# Autodesk Inventor assembly: elevation_assembly_blacha_gieta
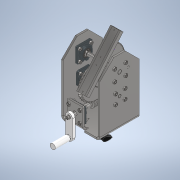
[picture p0: Inventor's stored thumbnail of the model, 180x180]
Saved by Autodesk Inventor 2020 (Build 240168000, 168)
## iProperties
Created: 2020-08-26
Part Number: elevation_assembly_blacha_gieta
Document SubType Name: Assembly
Designer: Hesekiel
Author: Hesekiel
## Documents named in this file (43)
- C:\Users\Hesekiel\Desktop\Equatorial-Mount-MUM\Mechanika\Mechanizm elewacji Filip\CAD\elevation_assembly_blacha_gieta.iam
- C:\Users\Hesekiel\Desktop\Equatorial-Mount-MUM\Mechanika\Mechanizm elewacji Filip\CAD\baza_blacha_gięta.ipt
- C:\Users\Hesekiel\Desktop\Equatorial-Mount-MUM\Mechanika\Mechanizm elewacji Filip\CAD\F4BSS 20M-YTPSS\F4BSS 20M-YTPSS.iam
- C:\Users\Hesekiel\Desktop\Equatorial-Mount-MUM\Mechanika\Mechanizm elewacji Filip\CAD\FY 15 FM\FY 15 FM.iam
- C:\Users\Hesekiel\Desktop\Equatorial-Mount-MUM\Mechanika\Mechanizm elewacji Filip\CAD\elevation_assembly_blacha_gieta\Design Accelerator\Bolted Connection4.iam
- C:\Users\Hesekiel\Desktop\Equatorial-Mount-MUM\Mechanika\Mechanizm elewacji Filip\CAD\elevation_assembly_blacha_gieta\Design Accelerator\Bolted Connection5.iam
- C:\Users\Hesekiel\Desktop\Equatorial-Mount-MUM\Mechanika\Mechanizm elewacji Filip\CAD\elevation_assembly_blacha_gieta\Design Accelerator\Bolted Connection6.iam
- C:\Users\Hesekiel\Desktop\Equatorial-Mount-MUM\Mechanika\Mechanizm elewacji Filip\CAD\elevation_assembly_blacha_gieta\Design Accelerator\Bolted Connection7.iam
- C:\Users\Hesekiel\Desktop\Equatorial-Mount-MUM\Mechanika\Mechanizm elewacji Filip\CAD\elevation_assembly_blacha_gieta\Design Accelerator\Bolted Connection8.iam
- C:\Users\Hesekiel\Desktop\Equatorial-Mount-MUM\Mechanika\Mechanizm elewacji Filip\CAD\elevation_assembly_blacha_gieta\Design Accelerator\Bolted Connection9.iam
- C:\Users\Hesekiel\Desktop\Equatorial-Mount-MUM\Mechanika\Mechanizm elewacji Filip\CAD\elevation_assembly_blacha_gieta\Design Accelerator\Bolted Connection10.iam
- C:\Users\Hesekiel\Desktop\Equatorial-Mount-MUM\Mechanika\Mechanizm elewacji Filip\CAD\elevation_assembly_blacha_gieta\Design Accelerator\Bolted Connection11.iam
- C:\Users\Hesekiel\Desktop\Equatorial-Mount-MUM\Mechanika\Mechanizm elewacji Filip\CAD\elevation_assembly_blacha_gieta\Design Accelerator\Bolted Connection12.iam
- C:\Users\Hesekiel\Desktop\Equatorial-Mount-MUM\Mechanika\Mechanizm elewacji Filip\CAD\elevation_assembly_blacha_gieta\Design Accelerator\Bolted Connection13.iam
- C:\Users\Hesekiel\Desktop\Equatorial-Mount-MUM\Mechanika\Mechanizm elewacji Filip\CAD\elevation_assembly_blacha_gieta\Design Accelerator\Bolted Connection14.iam
- C:\Users\Hesekiel\Desktop\Equatorial-Mount-MUM\Mechanika\Mechanizm elewacji Filip\CAD\elevation_assembly_blacha_gieta\Design Accelerator\Bolted Connection15.iam
- C:\Users\Hesekiel\Desktop\Equatorial-Mount-MUM\Mechanika\Mechanizm elewacji Filip\CAD\elevation_assembly_blacha_gieta\Design Accelerator\Bolted Connection16.iam
- C:\Users\Hesekiel\Desktop\Equatorial-Mount-MUM\Mechanika\Mechanizm elewacji Filip\CAD\elevation_assembly_blacha_gieta\Design Accelerator\Bolted Connection17.iam
- C:\Users\Hesekiel\Desktop\Equatorial-Mount-MUM\Mechanika\Mechanizm elewacji Filip\CAD\elevation_assembly_blacha_gieta\Design Accelerator\Bolted Connection18.iam
- C:\Users\Hesekiel\Desktop\Equatorial-Mount-MUM\Mechanika\Mechanizm elewacji Filip\CAD\elevation_assembly_blacha_gieta\Design Accelerator\Bolted Connection19.iam
- C:\Users\Hesekiel\Desktop\Equatorial-Mount-MUM\Mechanika\Mechanizm elewacji Filip\CAD\elevation_assembly_blacha_gieta\Design Accelerator\Bolted Connection20.iam
- C:\Users\Hesekiel\Desktop\Equatorial-Mount-MUM\Mechanika\Mechanizm elewacji Filip\CAD\elevation_assembly_blacha_gieta\Design Accelerator\Bolted Connection21.iam
- C:\Users\Hesekiel\Desktop\Equatorial-Mount-MUM\Mechanika\Mechanizm elewacji Filip\CAD\elevation_assembly_blacha_gieta\Design Accelerator\Bolted Connection22.iam
- C:\Users\Hesekiel\Desktop\Equatorial-Mount-MUM\Mechanika\Mechanizm elewacji Filip\CAD\elevation_assembly_blacha_gieta\Design Accelerator\Bolted Connection23.iam
- C:\Users\Hesekiel\Desktop\Equatorial-Mount-MUM\Mechanika\Mechanizm elewacji Filip\CAD\elevation_assembly_blacha_gieta\Design Accelerator\Bolted Connection24.iam
- C:\Users\Hesekiel\Desktop\Equatorial-Mount-MUM\Mechanika\Mechanizm elewacji Filip\CAD\elevation_assembly_blacha_gieta\Design Accelerator\Bolted Connection25.iam
- C:\Users\Hesekiel\Desktop\Equatorial-Mount-MUM\Mechanika\Mechanizm elewacji Filip\CAD\elevation_assembly_blacha_gieta\Design Accelerator\Bolted Connection26.iam
- C:\Users\Hesekiel\Desktop\Equatorial-Mount-MUM\Mechanika\Mechanizm elewacji Filip\CAD\elevation_assembly_blacha_gieta\Design Accelerator\Bolted Connection27.iam
- C:\Users\Hesekiel\Desktop\Equatorial-Mount-MUM\Mechanika\Mechanizm elewacji Filip\CAD\wał_półkola.ipt
- C:\Users\Hesekiel\Desktop\Equatorial-Mount-MUM\Mechanika\Mechanizm elewacji Filip\CAD\worm_gear.iam
- C:\Users\Hesekiel\Desktop\Equatorial-Mount-MUM\Mechanika\Mechanizm elewacji Filip\CAD\rack_and_pinion.iam
- C:\Users\Hesekiel\Desktop\Equatorial-Mount-MUM\Mechanika\Mechanizm elewacji Filip\CAD\wał_uzębienia.ipt
- C:\Users\Hesekiel\Desktop\Equatorial-Mount-MUM\Mechanika\Mechanizm elewacji Filip\CAD\ramię_korby.ipt
- C:\Users\Hesekiel\Desktop\Equatorial-Mount-MUM\Mechanika\Mechanizm elewacji Filip\CAD\rączka_korby.ipt
- C:\Users\Hesekiel\Desktop\Equatorial-Mount-MUM\Mechanika\Mechanizm elewacji Filip\CAD\elevation_assembly_blacha_gieta\Design Accelerator\Bolted Connection28.iam
- C:\Users\Hesekiel\Desktop\Equatorial-Mount-MUM\Mechanika\Mechanizm elewacji Filip\CAD\elevation_assembly_blacha_gieta\Design Accelerator\Bolted Connection29.iam
- C:\Users\Hesekiel\Desktop\Equatorial-Mount-MUM\Mechanika\Uchwyty, elementy i inne\szyna.ipt
- C:\Users\Hesekiel\Desktop\Equatorial-Mount-MUM\Mechanika\Mechanizm elewacji Filip\CAD\uchwyt_szyny.ipt
- C:\Users\Hesekiel\Desktop\Equatorial-Mount-MUM\Mechanika\Mechanizm elewacji Filip\CAD\elevation_assembly_blacha_gieta\Design Accelerator\Bolted Connection31.iam
- C:\Users\Hesekiel\Desktop\Equatorial-Mount-MUM\Mechanika\Mechanizm elewacji Filip\CAD\elevation_assembly_blacha_gieta\Design Accelerator\Bolted Connection32.iam
- C:\Users\Hesekiel\Desktop\Equatorial-Mount-MUM\Mechanika\Mechanizm elewacji Filip\CAD\elevation_assembly_blacha_gieta\Design Accelerator\Bolted Connection33.iam
- C:\Users\Hesekiel\Desktop\Equatorial-Mount-MUM\Mechanika\Mechanizm elewacji Filip\CAD\manfrotto-494rc2-tripod-head.snapshot.1\Manfrotto 494RC2 - Tripod Head\Manfrotto - 494RC2 Head Assy.iam
- C:\Users\Hesekiel\Desktop\Equatorial-Mount-MUM\Mechanika\Mechanizm elewacji Filip\CAD\M6x6_DIN914.ipt
## Components (48 placed, 14 different names)
1. baza_blacha_gięta:1 — Flush:1, Mate:1, Mate:2, Mate:3, Mate:4, Mate:5, Mate:6, Mate:7, Mate:21, Mate:22, Mate:23, Mate:24, Mate:25, Mate:26, Mate:27, Mate:28, Mate:29, Mate:30, Mate:31, Mate:32, Rotational:2, Angle:1, Rotational:3, Angle:2, Rotational:4, Mate:101, Mate:102
2. F4BSS 20M-YTPSS:1 [sub-assembly] — Mate:2, Mate:3, Mate:4, Mate:57, Mate:58, Mate:59, Mate:60, Mate:61, Mate:62, Mate:63, Mate:64
3. F4BSS 20M-YTPSS:2 [sub-assembly] — Mate:5, Mate:6, Mate:7, Mate:49, Mate:50, Mate:51, Mate:52, Mate:53, Mate:54, Mate:55, Mate:56
4. FY 15 FM:1 [sub-assembly] — Mate:21, Mate:22, Mate:23, Mate:41, Mate:42, Mate:43, Mate:44, Mate:45, Mate:46, Mate:47, Mate:48
5. FY 15 FM:2 [sub-assembly] — Mate:24, Mate:25, Mate:26, Mate:73, Mate:74, Mate:75, Mate:76, Mate:77, Mate:78, Mate:79, Mate:80
6. F4BSS 20M-YTPSS:3 [sub-assembly] — Mate:30, Mate:31, Mate:32, Mate:65, Mate:66, Mate:67, Mate:68, Mate:69, Mate:70, Mate:71, Mate:72
7. F4BSS 20M-YTPSS:4 [sub-assembly] — Mate:27, Mate:28, Mate:29, Mate:33, Mate:34, Mate:35, Mate:36, Mate:37, Mate:38, Mate:39, Mate:40
8. Bolted Connection:1 [sub-assembly] — Mate:33, Mate:34
9. Bolted Connection:2 [sub-assembly] — Mate:35, Mate:36
10. Bolted Connection:3 [sub-assembly] — Mate:37, Mate:38
11. Bolted Connection:4 [sub-assembly] — Mate:39, Mate:40
12. Bolted Connection:5 [sub-assembly] — Mate:41, Mate:42
13. Bolted Connection:6 [sub-assembly] — Mate:43, Mate:44
14. Bolted Connection:7 [sub-assembly] — Mate:45, Mate:46
15. Bolted Connection:8 [sub-assembly] — Mate:47, Mate:48
16. Bolted Connection:9 [sub-assembly] — Mate:49, Mate:50
17. Bolted Connection:10 [sub-assembly] — Mate:51, Mate:52
18. Bolted Connection:11 [sub-assembly] — Mate:53, Mate:54
19. Bolted Connection:12 [sub-assembly] — Mate:55, Mate:56
20. Bolted Connection:13 [sub-assembly] — Mate:57, Mate:58
21. Bolted Connection:14 [sub-assembly] — Mate:59, Mate:60
22. Bolted Connection:15 [sub-assembly] — Mate:61, Mate:62
23. Bolted Connection:16 [sub-assembly] — Mate:63, Mate:64
24. Bolted Connection:17 [sub-assembly] — Mate:65, Mate:66
25. Bolted Connection:18 [sub-assembly] — Mate:67, Mate:68
26. Bolted Connection:19 [sub-assembly] — Mate:69, Mate:70
27. Bolted Connection:20 [sub-assembly] — Mate:71, Mate:72
28. Bolted Connection:21 [sub-assembly] — Mate:73, Mate:74
29. Bolted Connection:22 [sub-assembly] — Mate:75, Mate:76
30. Bolted Connection:23 [sub-assembly] — Mate:77, Mate:78
31. Bolted Connection:24 [sub-assembly] — Mate:79, Mate:80
32. wał_półkola:1 — Rotational:2, Angle:1, Mate:81, Mate:107
33. rack_and_pinion:1 [sub-assembly] — Mate:81, Mate:82, Mate:84, Mate:92, Mate:93, Mate:94, Mate:104, Mate:108
34. worm_gear:1 [sub-assembly] — Mate:83, Mate:84, Rotational:4, Rigid:6, Mate:106
35. wał_uzębienia:1 — Rotational:3, Angle:2, Mate:82, Mate:83, Mate:103, Mate:105
36. ramię_korby:1 — Rigid:6, Rigid:7, Mate:85, Mate:86, Mate:87, Mate:88
37. rączka_korby:1 — Rigid:7
38. Bolted Connection:25 [sub-assembly] — Mate:85, Mate:86
39. Bolted Connection:26 [sub-assembly] — Mate:87, Mate:88
40. uchwyt_szyny:1 — Flush:2, Mate:89, Mate:90, Mate:91, Mate:92, Mate:93, Mate:94, Mate:95, Mate:96, Mate:97, Mate:98, Mate:99, Mate:100
41. Bolted Connection:27 [sub-assembly] — Mate:95, Mate:96
42. Bolted Connection:28 [sub-assembly] — Mate:97, Mate:98
43. Bolted Connection:29 [sub-assembly] — Mate:99, Mate:100
44. szyna:1 — Flush:2, Mate:89, Mate:90, Mate:91
45. Manfrotto - 494RC2 Head Assy:1 [sub-assembly] — Mate:101, Mate:102
46. M6x6_DIN914:1 — Mate:103, Mate:104
47. M6x6_DIN914:2 — Mate:105, Mate:106
48. M6x6_DIN914:3 — Mate:107, Mate:108
## Relationships (104: Mate 95, RevoluteJoint 3, Flush 2, Angle 2, WeldJoint 2)
- Flush:1: baza_blacha_gięta:1
- Mate:1: baza_blacha_gięta:1
- Mate:2: baza_blacha_gięta:1 ↔ F4BSS 20M-YTPSS:1
- Mate:3: baza_blacha_gięta:1 ↔ F4BSS 20M-YTPSS:1
- Mate:4: baza_blacha_gięta:1 ↔ F4BSS 20M-YTPSS:1
- Mate:5: baza_blacha_gięta:1 ↔ F4BSS 20M-YTPSS:2
- Mate:6: baza_blacha_gięta:1 ↔ F4BSS 20M-YTPSS:2
- Mate:7: baza_blacha_gięta:1 ↔ F4BSS 20M-YTPSS:2
- Mate:21: baza_blacha_gięta:1 ↔ FY 15 FM:1
- Mate:22: baza_blacha_gięta:1 ↔ FY 15 FM:1
- Mate:23: baza_blacha_gięta:1 ↔ FY 15 FM:1
- Mate:24: baza_blacha_gięta:1 ↔ FY 15 FM:2
- Mate:25: baza_blacha_gięta:1 ↔ FY 15 FM:2
- Mate:26: baza_blacha_gięta:1 ↔ FY 15 FM:2
- Mate:27: baza_blacha_gięta:1 ↔ F4BSS 20M-YTPSS:4
- Mate:28: baza_blacha_gięta:1 ↔ F4BSS 20M-YTPSS:4
- Mate:29: baza_blacha_gięta:1 ↔ F4BSS 20M-YTPSS:4
- Mate:30: baza_blacha_gięta:1 ↔ F4BSS 20M-YTPSS:3
- Mate:31: baza_blacha_gięta:1 ↔ F4BSS 20M-YTPSS:3
- Mate:32: baza_blacha_gięta:1 ↔ F4BSS 20M-YTPSS:3
- Mate:33: F4BSS 20M-YTPSS:4 ↔ Bolted Connection:1
- Mate:34: F4BSS 20M-YTPSS:4 ↔ Bolted Connection:1
- Mate:35: F4BSS 20M-YTPSS:4 ↔ Bolted Connection:2
- Mate:36: F4BSS 20M-YTPSS:4 ↔ Bolted Connection:2
- Mate:37: F4BSS 20M-YTPSS:4 ↔ Bolted Connection:3
- Mate:38: F4BSS 20M-YTPSS:4 ↔ Bolted Connection:3
- Mate:39: F4BSS 20M-YTPSS:4 ↔ Bolted Connection:4
- Mate:40: F4BSS 20M-YTPSS:4 ↔ Bolted Connection:4
- Mate:41: FY 15 FM:1 ↔ Bolted Connection:5
- Mate:42: FY 15 FM:1 ↔ Bolted Connection:5
- Mate:43: FY 15 FM:1 ↔ Bolted Connection:6
- Mate:44: FY 15 FM:1 ↔ Bolted Connection:6
- Mate:45: FY 15 FM:1 ↔ Bolted Connection:7
- Mate:46: FY 15 FM:1 ↔ Bolted Connection:7
- Mate:47: FY 15 FM:1 ↔ Bolted Connection:8
- Mate:48: FY 15 FM:1 ↔ Bolted Connection:8
- Mate:49: F4BSS 20M-YTPSS:2 ↔ Bolted Connection:9
- Mate:50: F4BSS 20M-YTPSS:2 ↔ Bolted Connection:9
- Mate:51: F4BSS 20M-YTPSS:2 ↔ Bolted Connection:10
- Mate:52: F4BSS 20M-YTPSS:2 ↔ Bolted Connection:10
- Mate:53: F4BSS 20M-YTPSS:2 ↔ Bolted Connection:11
- Mate:54: F4BSS 20M-YTPSS:2 ↔ Bolted Connection:11
- Mate:55: F4BSS 20M-YTPSS:2 ↔ Bolted Connection:12
- Mate:56: F4BSS 20M-YTPSS:2 ↔ Bolted Connection:12
- Mate:57: F4BSS 20M-YTPSS:1 ↔ Bolted Connection:13
- Mate:58: F4BSS 20M-YTPSS:1 ↔ Bolted Connection:13
- Mate:59: F4BSS 20M-YTPSS:1 ↔ Bolted Connection:14
- Mate:60: F4BSS 20M-YTPSS:1 ↔ Bolted Connection:14
- Mate:61: F4BSS 20M-YTPSS:1 ↔ Bolted Connection:15
- Mate:62: F4BSS 20M-YTPSS:1 ↔ Bolted Connection:15
- Mate:63: F4BSS 20M-YTPSS:1 ↔ Bolted Connection:16
- Mate:64: F4BSS 20M-YTPSS:1 ↔ Bolted Connection:16
- Mate:65: F4BSS 20M-YTPSS:3 ↔ Bolted Connection:17
- Mate:66: F4BSS 20M-YTPSS:3 ↔ Bolted Connection:17
- Mate:67: F4BSS 20M-YTPSS:3 ↔ Bolted Connection:18
- Mate:68: F4BSS 20M-YTPSS:3 ↔ Bolted Connection:18
- Mate:69: F4BSS 20M-YTPSS:3 ↔ Bolted Connection:19
- Mate:70: F4BSS 20M-YTPSS:3 ↔ Bolted Connection:19
- Mate:71: F4BSS 20M-YTPSS:3 ↔ Bolted Connection:20
- Mate:72: F4BSS 20M-YTPSS:3 ↔ Bolted Connection:20
- Mate:73: FY 15 FM:2 ↔ Bolted Connection:21
- Mate:74: FY 15 FM:2 ↔ Bolted Connection:21
- Mate:75: FY 15 FM:2 ↔ Bolted Connection:22
- Mate:76: FY 15 FM:2 ↔ Bolted Connection:22
- Mate:77: FY 15 FM:2 ↔ Bolted Connection:23
- Mate:78: FY 15 FM:2 ↔ Bolted Connection:23
- Mate:79: FY 15 FM:2 ↔ Bolted Connection:24
- Mate:80: FY 15 FM:2 ↔ Bolted Connection:24
- Rotational:2 [RevoluteJoint]: baza_blacha_gięta:1 ↔ wał_półkola:1
- Angle:1 (0 deg): baza_blacha_gięta:1 ↔ wał_półkola:1
- Rotational:3 [RevoluteJoint]: baza_blacha_gięta:1 ↔ wał_uzębienia:1
- Angle:2 (0 deg): baza_blacha_gięta:1 ↔ wał_uzębienia:1
- Mate:81: wał_półkola:1 ↔ rack_and_pinion:1
- Mate:82: rack_and_pinion:1 ↔ wał_uzębienia:1
- Mate:83: worm_gear:1 ↔ wał_uzębienia:1
- Mate:84 (10 mm): rack_and_pinion:1 ↔ worm_gear:1
- Rotational:4 [RevoluteJoint]: baza_blacha_gięta:1 ↔ worm_gear:1
- Rigid:6 [WeldJoint]: worm_gear:1 ↔ ramię_korby:1
- Rigid:7 [WeldJoint]: ramię_korby:1 ↔ rączka_korby:1
- Mate:85: ramię_korby:1 ↔ Bolted Connection:25
- Mate:86: ramię_korby:1 ↔ Bolted Connection:25
- Mate:87: ramię_korby:1 ↔ Bolted Connection:26
- Mate:88: ramię_korby:1 ↔ Bolted Connection:26
- Flush:2: uchwyt_szyny:1 ↔ szyna:1
- Mate:89: uchwyt_szyny:1 ↔ szyna:1
- Mate:90: uchwyt_szyny:1 ↔ szyna:1
- Mate:91: uchwyt_szyny:1 ↔ szyna:1
- Mate:92: rack_and_pinion:1 ↔ uchwyt_szyny:1
- Mate:93: rack_and_pinion:1 ↔ uchwyt_szyny:1
- Mate:94: rack_and_pinion:1 ↔ uchwyt_szyny:1
- Mate:95: uchwyt_szyny:1 ↔ Bolted Connection:27
- Mate:96: uchwyt_szyny:1 ↔ Bolted Connection:27
- Mate:97: uchwyt_szyny:1 ↔ Bolted Connection:28
- Mate:98: uchwyt_szyny:1 ↔ Bolted Connection:28
- Mate:99: uchwyt_szyny:1 ↔ Bolted Connection:29
- Mate:100: uchwyt_szyny:1 ↔ Bolted Connection:29
- Mate:101: baza_blacha_gięta:1 ↔ Manfrotto - 494RC2 Head Assy:1
- Mate:102: baza_blacha_gięta:1 ↔ Manfrotto - 494RC2 Head Assy:1
- Mate:103: wał_uzębienia:1 ↔ M6x6_DIN914:1
- Mate:104: rack_and_pinion:1 ↔ M6x6_DIN914:1
- Mate:105: wał_uzębienia:1 ↔ M6x6_DIN914:2
- Mate:106: worm_gear:1 ↔ M6x6_DIN914:2
- Mate:107: wał_półkola:1 ↔ M6x6_DIN914:3
- Mate:108: rack_and_pinion:1 ↔ M6x6_DIN914:3
